# Autodesk Inventor assembly: Robot Assembly 2
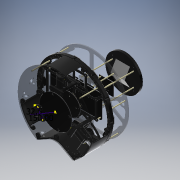
[picture p0: Inventor's stored thumbnail of the model, 180x180]
Saved by Autodesk Inventor 2018 (Build 220112000, 112)
## iProperties
Created: 2018-07-12
Part Number: Robot Assembly 2
Document SubType Name: Assembly
Designer: matth
Author: matth
## Documents named in this file (20)
- C:\Users\matth\Dropbox\M&A\Robotics-2018\Design and Hardware\Maxon Parts\Robot Assembly 2.iam
- C:\Users\matth\Dropbox\M&A\Robotics-2018\Design and Hardware\Maxon Parts\Base Plate.ipt
- C:\Users\matth\Dropbox\M&A\Robotics-2018\Design and Hardware\Maxon Parts\Capture Zone.ipt
- C:\Users\matth\Dropbox\M&A\Robotics-2018\Design and Hardware\Maxon Parts\Wheel Guard.ipt
- C:\Users\matth\Dropbox\M&A\Robotics-2018\Design and Hardware\Maxon Parts\Maxon Mount.ipt
- C:\Users\matth\Dropbox\M&A\Robotics-2018\Design and Hardware\Maxon Parts\50mm Standoff.ipt
- C:\Users\matth\Dropbox\M&A\Robotics-2018\Design and Hardware\Maxon Parts\TSSP Ring.ipt
- C:\Users\matth\Dropbox\M&A\Robotics-2018\Design and Hardware\Maxon Parts\40mm Standoff.ipt
- C:\Users\matth\Dropbox\M&A\Robotics-2018\Design and Hardware\Maxon Parts\Top Plate.ipt
- C:\Users\matth\Dropbox\M&A\Robotics-2018\Design and Hardware\Maxon Parts\10mm Standoff.ipt
- C:\Users\matth\Dropbox\M&A\Robotics-2018\Design and Hardware\Maxon Parts\Pixy Bracket.ipt
- C:\Users\matth\Dropbox\M&A\Robotics-2018\Design and Hardware\Maxon Parts\20mm Standoff.ipt
- C:\Users\matth\Dropbox\M&A\Robotics-2018\Design and Hardware\Maxon Parts\87.5mm Standoff.ipt
- C:\Users\matth\Dropbox\M&A\Robotics-2018\Design and Hardware\Maxon Parts\Mirror Mount.ipt
- C:\Users\matth\Dropbox\M&A\Robotics-2018\Design and Hardware\Maxon Parts\Pixy Sketch.ipt
- C:\Users\matth\Dropbox\M&A\Robotics-2018\Design and Hardware\Render Parts\TSSP Board.ipt
- C:\Users\matth\Dropbox\M&A\Robotics-2018\Design and Hardware\Render Parts\Light Sensor.ipt
- C:\Users\matth\Dropbox\M&A\Robotics-2018\Design and Hardware\Render Parts\TSSP Receiver.ipt
- C:\Users\matth\Dropbox\M&A\Robotics-2018\Design and Hardware\Render Parts\Teensy And Breakout.ipt
- C:\Users\matth\Dropbox\M&A\Robotics-2018\Design and Hardware\Render Parts\Power Supply.ipt
## Components (59 placed, 19 different names)
1. Capture Zone:1 — Mate:1
2. Base Plate:1 — Mate:1, Mate:2, Mate:3, Mate:4, Mate:5, Mate:6, Mate:7, Mate:8, Mate:9, Mate:10, Mate:11, Mate:12, Mate:13, Mate:14, Mate:66
3. Maxon Mount:1 — Mate:2
4. Maxon Mount:2 — Mate:5, Mate:6
5. Maxon Mount:3 — Mate:3, Mate:4
6. Wheel Guard:1 — Mate:7
7. Wheel Guard:2 — Mate:8, Mate:9, Mate:10
8. Wheel Guard:3 — Mate:11, Mate:12, Mate:15
9. 50mm Standoff:1 — Mate:14
10. 50mm Standoff:2 — Mate:13
11. TSSP Ring:1 — Mate:15, Mate:16, Mate:17, Mate:18, Mate:19, Mate:20, Mate:21, Mate:39, Mate:40, Mate:41, Mate:42, Mate:43, Mate:44, Mate:45, Mate:46, Mate:47, Mate:48, Mate:49, Mate:50, Mate:51, Mate:52, Mate:53, Mate:54, Mate:55, Mate:56, Mate:57, Mate:58, Mate:59, Mate:60, Mate:61, Mate:62, Mate:63, Mate:64, Mate:65, Mate:67, Mate:68, Mate:69, Mate:74, Mate:75, Mate:76, Mate:77
12. 40mm Standoff:1 — Mate:17
13. 40mm Standoff:2 — Mate:20
14. 40mm Standoff:3 — Mate:21
15. 40mm Standoff:4 — Mate:19
16. 40mm Standoff:5 — Mate:16
17. 40mm Standoff:6 — Mate:18, Mate:22
18. Top Plate:1 — Mate:22, Mate:23, Mate:24, Mate:25, Mate:26, Mate:31, Mate:32, Mate:33, Mate:34
19. 10mm Standoff:1 — Mate:26, Mate:27
20. 10mm Standoff:2 — Mate:25
21. 10mm Standoff:3 — Mate:24
22. 10mm Standoff:4 — Mate:23
23. Pixy Bracket:1 — Mate:27, Mate:28, Mate:29, Mate:30
24. 20mm Standoff:1 — Mate:28, Mate:38
25. 20mm Standoff:2 — Mate:29, Mate:36
26. 20mm Standoff:3 — Mate:30, Mate:37
27. 87.5mm Standoff:1 — Mate:31
28. 87.5mm Standoff:2 — Mate:32
29. 87.5mm Standoff:3 — Mate:33
30. 87.5mm Standoff:4 — Mate:34, Mate:35
31. Mirror Mount:1 — Mate:35
32. Pixy Sketch:1 — Mate:36, Mate:37, Mate:38
33. 10mm Standoff:5 — Mate:39, Mate:72
34. 10mm Standoff:6 — Mate:40, Mate:73
35. 10mm Standoff:7 — Mate:41
36. 10mm Standoff:8 — Mate:42
37. TSSP Board:1 — Mate:58, Mate:59
38. TSSP Board:2 — Mate:62, Mate:63
39. TSSP Board:3 — Mate:54, Mate:55
40. TSSP Board:4 — Mate:64, Mate:65
41. TSSP Board:5 — Mate:43, Mate:44
42. TSSP Board:6 — Mate:47, Mate:48
43. TSSP Board:7 — Mate:45, Mate:46
44. TSSP Board:8 — Mate:49, Mate:50
45. TSSP Board:9 — Mate:51
46. TSSP Board:10 — Mate:52, Mate:53
47. TSSP Board:11 — Mate:60, Mate:61
48. TSSP Board:12 — Mate:56, Mate:57
49. Light Sensor:1 — Mate:66
50. 10mm Standoff:9 — Mate:67
51. 10mm Standoff:10 — Mate:69, Mate:71
52. 10mm Standoff:11 — Mate:68, Mate:70
53. TSSP Receiver:1 — Mate:70, Mate:71
54. Teensy And Breakout:1 — Mate:72, Mate:73
55. 10mm Standoff:12 — Mate:77
56. 10mm Standoff:13 — Mate:74, Mate:78
57. 10mm Standoff:14 — Mate:76
58. 10mm Standoff:15 — Mate:75
59. Power Supply:1 — Mate:78
## Relationships (78: Mate 78)
- Mate:1: Capture Zone:1 ↔ Base Plate:1
- Mate:2: Base Plate:1 ↔ Maxon Mount:1
- Mate:3: Base Plate:1 ↔ Maxon Mount:3
- Mate:4: Base Plate:1 ↔ Maxon Mount:3
- Mate:5: Base Plate:1 ↔ Maxon Mount:2
- Mate:6: Base Plate:1 ↔ Maxon Mount:2
- Mate:7: Base Plate:1 ↔ Wheel Guard:1
- Mate:8: Base Plate:1 ↔ Wheel Guard:2
- Mate:9: Base Plate:1 ↔ Wheel Guard:2
- Mate:10: Base Plate:1 ↔ Wheel Guard:2
- Mate:11: Base Plate:1 ↔ Wheel Guard:3
- Mate:12: Base Plate:1 ↔ Wheel Guard:3
- Mate:13: Base Plate:1 ↔ 50mm Standoff:2
- Mate:14: Base Plate:1 ↔ 50mm Standoff:1
- Mate:15: Wheel Guard:3 ↔ TSSP Ring:1
- Mate:16: TSSP Ring:1 ↔ 40mm Standoff:5
- Mate:17: TSSP Ring:1 ↔ 40mm Standoff:1
- Mate:18: TSSP Ring:1 ↔ 40mm Standoff:6
- Mate:19: TSSP Ring:1 ↔ 40mm Standoff:4
- Mate:20: TSSP Ring:1 ↔ 40mm Standoff:2
- Mate:21: TSSP Ring:1 ↔ 40mm Standoff:3
- Mate:22: 40mm Standoff:6 ↔ Top Plate:1
- Mate:23: Top Plate:1 ↔ 10mm Standoff:4
- Mate:24: Top Plate:1 ↔ 10mm Standoff:3
- Mate:25: Top Plate:1 ↔ 10mm Standoff:2
- Mate:26: Top Plate:1 ↔ 10mm Standoff:1
- Mate:27: 10mm Standoff:1 ↔ Pixy Bracket:1
- Mate:28: Pixy Bracket:1 ↔ 20mm Standoff:1
- Mate:29: Pixy Bracket:1 ↔ 20mm Standoff:2
- Mate:30: Pixy Bracket:1 ↔ 20mm Standoff:3
- Mate:31: Top Plate:1 ↔ 87.5mm Standoff:1
- Mate:32: Top Plate:1 ↔ 87.5mm Standoff:2
- Mate:33: Top Plate:1 ↔ 87.5mm Standoff:3
- Mate:34: Top Plate:1 ↔ 87.5mm Standoff:4
- Mate:35: 87.5mm Standoff:4 ↔ Mirror Mount:1
- Mate:36: 20mm Standoff:2 ↔ Pixy Sketch:1
- Mate:37: 20mm Standoff:3 ↔ Pixy Sketch:1
- Mate:38: 20mm Standoff:1 ↔ Pixy Sketch:1
- Mate:39: TSSP Ring:1 ↔ 10mm Standoff:5
- Mate:40: TSSP Ring:1 ↔ 10mm Standoff:6
- Mate:41: TSSP Ring:1 ↔ 10mm Standoff:7
- Mate:42: TSSP Ring:1 ↔ 10mm Standoff:8
- Mate:43: TSSP Ring:1 ↔ TSSP Board:5
- Mate:44: TSSP Ring:1 ↔ TSSP Board:5
- Mate:45: TSSP Ring:1 ↔ TSSP Board:7
- Mate:46: TSSP Ring:1 ↔ TSSP Board:7
- Mate:47: TSSP Ring:1 ↔ TSSP Board:6
- Mate:48: TSSP Ring:1 ↔ TSSP Board:6
- Mate:49: TSSP Ring:1 ↔ TSSP Board:8
- Mate:50: TSSP Ring:1 ↔ TSSP Board:8
- Mate:51: TSSP Ring:1 ↔ TSSP Board:9
- Mate:52: TSSP Ring:1 ↔ TSSP Board:10
- Mate:53: TSSP Ring:1 ↔ TSSP Board:10
- Mate:54: TSSP Ring:1 ↔ TSSP Board:3
- Mate:55: TSSP Ring:1 ↔ TSSP Board:3
- Mate:56: TSSP Ring:1 ↔ TSSP Board:12
- Mate:57: TSSP Ring:1 ↔ TSSP Board:12
- Mate:58: TSSP Ring:1 ↔ TSSP Board:1
- Mate:59: TSSP Ring:1 ↔ TSSP Board:1
- Mate:60: TSSP Ring:1 ↔ TSSP Board:11
- Mate:61: TSSP Ring:1 ↔ TSSP Board:11
- Mate:62: TSSP Ring:1 ↔ TSSP Board:2
- Mate:63: TSSP Ring:1 ↔ TSSP Board:2
- Mate:64: TSSP Ring:1 ↔ TSSP Board:4
- Mate:65: TSSP Ring:1 ↔ TSSP Board:4
- Mate:66: Base Plate:1 ↔ Light Sensor:1
- Mate:67: TSSP Ring:1 ↔ 10mm Standoff:9
- Mate:68: TSSP Ring:1 ↔ 10mm Standoff:11
- Mate:69: TSSP Ring:1 ↔ 10mm Standoff:10
- Mate:70: 10mm Standoff:11 ↔ TSSP Receiver:1
- Mate:71: 10mm Standoff:10 ↔ TSSP Receiver:1
- Mate:72: 10mm Standoff:5 ↔ Teensy And Breakout:1
- Mate:73: 10mm Standoff:6 ↔ Teensy And Breakout:1
- Mate:74: TSSP Ring:1 ↔ 10mm Standoff:13
- Mate:75: TSSP Ring:1 ↔ 10mm Standoff:15
- Mate:76: TSSP Ring:1 ↔ 10mm Standoff:14
- Mate:77: TSSP Ring:1 ↔ 10mm Standoff:12
- Mate:78: 10mm Standoff:13 ↔ Power Supply:1
